# Autodesk Inventor assembly: ASSY,ROBOT,2026
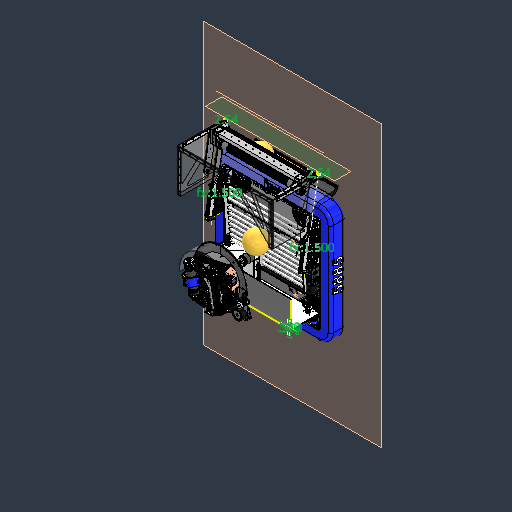
[picture p0: Inventor's stored thumbnail of the model, 512x512]
Saved by Autodesk Inventor 2026 (Build 300175050, 175E)
## iProperties
Created: 2026-01-24
Part Number: ASSY,ROBOT,2026
Document SubType Name: Assembly
Designer: Jthib
Mass: 66759.7 g
Surface Area: 127569 cm^2
Volume: 49905 cm^3
Density: 1.33774 g/cm^3
Author: Jthib
## Documents named in this file (14)
- C:\Users\Jthib\Documents\GitHub\2026-Robot-Mechanical\ASSY,ROBOT,2026.iam
- C:\Users\Jthib\Documents\GitHub\2026-Robot-Mechanical\Chassis\CHASSIS.iam
- C:\Users\Jthib\Documents\GitHub\2026-Robot-Mechanical\Spindexer\#Spindexer.iam
- C:\Users\Jthib\Documents\GitHub\2026-Robot-Mechanical\Shooter\Shooter - Front Motors\#SHOOTER.FRONT_MOTORS.iam
- C:\Users\Jthib\Documents\GitHub\2026-Robot-Mechanical\Shooter\Turret\#Turret.iam
- C:\Users\Jthib\Documents\GitHub\2026-Robot-Mechanical\#1_CAD Library\Power Transmission\Bearings\PURCHASED,HEX_BEARING.ipt
- C:\Users\Jthib\Documents\GitHub\2026-Robot-Mechanical\LINEAR_INTAKE\LINEAR_INTAKE_ASSY.iam
- C:\Users\Jthib\Documents\GitHub\2026-Robot-Mechanical\Chassis\Bumpers.ipt
- C:\Users\Jthib\Documents\GitHub\2026-Robot-Mechanical\Roller\ASSY.ROLLER.iam
- E:\Downloads\3DPRINT,BELT,GUARD\3DPRINT,BELT,GUARD\3DPRINT,BELT,GUARD.ipt
- C:\Users\Jthib\Documents\GitHub\2026-Robot-Mechanical\Spindexer\PURCHASED,20-1,90deg,MAX-PLANETARY.ipt
- C:\Users\Jthib\Documents\GitHub\2026-Robot-Mechanical\#1_CAD Library\Motors\MOTOR,REV,NEO,V1-1.ipt
- C:\Users\Jthib\Documents\GitHub\2026-Robot-Mechanical\LINEAR_INTAKE\INTAKE_EXT_PULLYS.ipt
- C:\Users\Jthib\Documents\GitHub\2026-Robot-Mechanical\LINEAR_INTAKE\55t_Belt.ipt
## Components (15 placed, 13 different names)
1. CHASSIS:1 [sub-assembly] — Flush:1, Flush:2, Flush:3, Mate:9, Mate:10, Flush:4, Flush:5, Mate:18, Flush:6, Flush:7, Insert:2, Flush:8, Mate:97, Mate:99, Mate:100, Flush:11, Flush:12, Mate:101, Mate:104
2. #Spindexer:1 [sub-assembly] — Mate:15, Mate:16, Mate:17, Flush:4, Flush:5, Mate:18, Flush:6, Flush:7, Mate:102
3. #SHOOTER.FRONT_MOTORS:1 [sub-assembly] — Mate:9, Mate:10, Insert:1, Mate:14
4. #Turret:1 [sub-assembly] — Insert:1, Mate:14, Mate:15, Mate:16, Mate:17
5. PURCHASED,HEX_BEARING:1 — Insert:2
6. Bumpers:1 — Mate:97, Mate:98, Mate:99
7. LINEAR_INTAKE_ASSY:2 [sub-assembly] — Mate:100, Flush:11, Flush:12, Mate:105, Mate:109, Mate:110
8. ASSY.ROLLER:1 [sub-assembly] — Mate:103
9. 3DPRINT,BELT,GUARD:1 — Mate:101, Mate:102
10. PURCHASED,20-1,90deg,MAX-PLANETARY:1 — Insert:3, Mate:103, Mate:104
11. MOTOR,REV,NEO,V1-1:1 — Insert:3
12. PURCHASED,HEX_BEARING:2 — Mate:105
13. INTAKE_EXT_PULLYS:1 — Mate:110, Mate:111
14. 55t_Belt:1 — Mate:111
15. INTAKE_EXT_PULLYS:2 — Mate:109
## Relationships (37: Mate 23, Flush 11, Insert 3)
- Flush:1 (-349.25 mm): CHASSIS:1
- Flush:2 (349.25 mm): CHASSIS:1
- Flush:3: CHASSIS:1
- Mate:9 (-190.5 mm): CHASSIS:1 ↔ #SHOOTER.FRONT_MOTORS:1
- Mate:10 (-190.5 mm): CHASSIS:1 ↔ #SHOOTER.FRONT_MOTORS:1
- Insert:1: #SHOOTER.FRONT_MOTORS:1 ↔ #Turret:1
- Mate:14: #SHOOTER.FRONT_MOTORS:1 ↔ #Turret:1
- Mate:15: #Spindexer:1 ↔ #Turret:1
- Mate:16: #Spindexer:1 ↔ #Turret:1
- Mate:17: #Spindexer:1 ↔ #Turret:1
- Flush:4: CHASSIS:1 ↔ #Spindexer:1
- Flush:5: CHASSIS:1 ↔ #Spindexer:1
- Mate:18: CHASSIS:1 ↔ #Spindexer:1
- Flush:6 (107.95 mm): CHASSIS:1 ↔ #Spindexer:1
- Flush:7: CHASSIS:1 ↔ #Spindexer:1
- Insert:2: CHASSIS:1 ↔ PURCHASED,HEX_BEARING:1
- Flush:8 (-100.0689 mm): CHASSIS:1
- Flush:10
- Mate:96 (165.6842 mm)
- Mate:97: CHASSIS:1 ↔ Bumpers:1
- Mate:98 (43.815 mm): Bumpers:1
- Mate:99: CHASSIS:1 ↔ Bumpers:1
- Mate:100: CHASSIS:1 ↔ LINEAR_INTAKE_ASSY:2
- Flush:11: CHASSIS:1 ↔ LINEAR_INTAKE_ASSY:2
- Flush:12: CHASSIS:1 ↔ LINEAR_INTAKE_ASSY:2
- Mate:101: CHASSIS:1 ↔ 3DPRINT,BELT,GUARD:1
- Mate:102 (82.55 mm): #Spindexer:1 ↔ 3DPRINT,BELT,GUARD:1
- Insert:3: PURCHASED,20-1,90deg,MAX-PLANETARY:1 ↔ MOTOR,REV,NEO,V1-1:1
- Mate:103 (12.7 mm): ASSY.ROLLER:1 ↔ PURCHASED,20-1,90deg,MAX-PLANETARY:1
- Mate:104 (-3.175 mm): CHASSIS:1 ↔ PURCHASED,20-1,90deg,MAX-PLANETARY:1
- Mate:105: LINEAR_INTAKE_ASSY:2 ↔ PURCHASED,HEX_BEARING:2
- [Mate]: 55t_Belt:1 ↔ INTAKE_EXT_PULLYS:2
- [Mate]: 55t_Belt:1 ↔ INTAKE_EXT_PULLYS:2
- [Mate]: INTAKE_EXT_PULLYS:1 ↔ 55t_Belt:1
- Mate:109: LINEAR_INTAKE_ASSY:2 ↔ INTAKE_EXT_PULLYS:2
- Mate:110: LINEAR_INTAKE_ASSY:2 ↔ INTAKE_EXT_PULLYS:1
- Mate:111: INTAKE_EXT_PULLYS:1 ↔ 55t_Belt:1
